# Autodesk Inventor assembly: Drive Roller Assembly 3 (Lexan)
(part 2 of 2)
- Mate:1213: Vex Pro 1x1 rectangular tubing 21.375 in length:1 ↔ Roller Crossbar Gusset (Custom):6
- Mate:1214: Vex Pro 1x1 rectangular tubing 14 in length (roller):1 ↔ Roller Crossbar Gusset (Custom):7
- Mate:1215: Vex Pro 1x1 rectangular tubing 14 in length (roller):1 ↔ Roller Crossbar Gusset (Custom):7
- Mate:1216: Vex Pro 1x1 rectangular tubing 14 in length (roller):1 ↔ Roller Crossbar Gusset (Custom):7
- Mate:1218: Vex Pro 1x1 rectangular tubing 14 in length:5 ↔ Bearing Mount Spacer 1-8 in:1
- Mate:1219: Vex Pro 1x1 rectangular tubing 14 in length:5 ↔ Bearing Mount Spacer 1-8 in:1
- Mate:1220: Vex Pro 1x1 rectangular tubing 14 in length:5 ↔ Bearing Mount Spacer 1-8 in:1
- Mate:1221: Vex Pro End Bearing Mount (Bolt):1 ↔ Bearing Mount Spacer 1-8 in:1
- Mate:1222: Vex Pro End Bearing Mount (Bolt):1 ↔ Bearing Mount Spacer 1-8 in:1
- Mate:1223: Vex Pro End Bearing Mount (Bolt):1 ↔ Bearing Mount Spacer 1-8 in:1
- Mate:1224: Vex Pro 1x1 rectangular tubing 14 in length:5 ↔ Bearing Mount Spacer 1-8 in:2
- Mate:1225: Vex Pro 1x1 rectangular tubing 14 in length:5 ↔ Bearing Mount Spacer 1-8 in:2
- Mate:1226: Vex Pro 1x1 rectangular tubing 14 in length:5 ↔ Bearing Mount Spacer 1-8 in:2
- Mate:1227: Vex Pro End Bearing Mount (Bolt):2 ↔ Bearing Mount Spacer 1-8 in:2
- Mate:1228: Vex Pro End Bearing Mount (Bolt):2 ↔ Bearing Mount Spacer 1-8 in:2
- Mate:1229: Vex Pro End Bearing Mount (Bolt):2 ↔ Bearing Mount Spacer 1-8 in:2
- Mate:1230: Vex Pro 1x1 rectangular tubing 14 in length:6 ↔ Bearing Mount Spacer 1-8 in:3
- Mate:1231: Vex Pro 1x1 rectangular tubing 14 in length:6 ↔ Bearing Mount Spacer 1-8 in:3
- Mate:1232: Vex Pro 1x1 rectangular tubing 14 in length:6 ↔ Bearing Mount Spacer 1-8 in:3
- Mate:1233: Vex Pro End Bearing Mount (Bolt):3 ↔ Bearing Mount Spacer 1-8 in:3
- Mate:1234: Vex Pro End Bearing Mount (Bolt):3 ↔ Bearing Mount Spacer 1-8 in:3
- Mate:1235: Vex Pro End Bearing Mount (Bolt):3 ↔ Bearing Mount Spacer 1-8 in:3
- Mate:1236: Vex Pro 1x1 rectangular tubing 14 in length:6 ↔ Bearing Mount Spacer 1-8 in:5
- Mate:1237: Vex Pro 1x1 rectangular tubing 14 in length:6 ↔ Bearing Mount Spacer 1-8 in:5
- Mate:1238: Vex Pro 1x1 rectangular tubing 14 in length:6 ↔ Bearing Mount Spacer 1-8 in:5
- Mate:1239: Vex Pro End Bearing Mount (Bolt):4 ↔ Bearing Mount Spacer 1-8 in:5
- Mate:1240: Vex Pro End Bearing Mount (Bolt):4 ↔ Bearing Mount Spacer 1-8 in:5
- Mate:1241: Vex Pro End Bearing Mount (Bolt):4 ↔ Bearing Mount Spacer 1-8 in:5
- Mate:1242: Hex Shaft Collar 3-8 in (7552K300):1 ↔ Hex Shaft 3-8 in (am-0855):3
- Mate:1243: Hex Shaft Collar 3-8 in (7552K300):1 ↔ Hex Shaft 3-8 in (am-0855):3
- Flush:41: Hex Shaft Collar 3-8 in (7552K300):1 ↔ Hex Shaft 3-8 in (am-0855):3
- Mate:1244: Hex Shaft Collar 3-8 in (7552K300):3 ↔ Hex Shaft 3-8 in (am-0855):4
- Mate:1245: Hex Shaft Collar 3-8 in (7552K300):3 ↔ Hex Shaft 3-8 in (am-0855):4
- Flush:42: Hex Shaft Collar 3-8 in (7552K300):3 ↔ Hex Shaft 3-8 in (am-0855):4
- Mate:1246: Vex Pro 1x1 rectangular tubing 14 in length:5 ↔ Vex Pro T gusset - OUT OF STOCK 1192014:3
- Mate:1247: Vex Pro 1x1 rectangular tubing 14 in length:5 ↔ Vex Pro T gusset - OUT OF STOCK 1192014:3
- Mate:1248: Vex Pro 1x1 rectangular tubing 14 in length:5 ↔ Vex Pro T gusset - OUT OF STOCK 1192014:3
- Mate:1249: Vex Pro 1x1 rectangular tubing 4 in length:1 ↔ Vex Pro T gusset - OUT OF STOCK 1192014:3
- Mate:1250: Vex Pro 1x1 rectangular tubing 14 in length:5 ↔ Vex Pro T gusset - OUT OF STOCK 1192014:4
- Mate:1251: Vex Pro 1x1 rectangular tubing 14 in length:5 ↔ Vex Pro T gusset - OUT OF STOCK 1192014:4
- Mate:1252: Vex Pro 1x1 rectangular tubing 14 in length:5 ↔ Vex Pro T gusset - OUT OF STOCK 1192014:4
- Mate:1253: Vex Pro 1x1 rectangular tubing 4 in length:1 ↔ Vex Pro T gusset - OUT OF STOCK 1192014:4
- Mate:1254: Vex Pro 1x1 rectangular tubing 14 in length:6 ↔ Vex Pro T gusset - OUT OF STOCK 1192014:5
- Mate:1255: Vex Pro 1x1 rectangular tubing 14 in length:6 ↔ Vex Pro T gusset - OUT OF STOCK 1192014:5
- Mate:1256: Vex Pro 1x1 rectangular tubing 14 in length:6 ↔ Vex Pro T gusset - OUT OF STOCK 1192014:5
- Mate:1257: Vex Pro 1x1 rectangular tubing 4 in length:2 ↔ Vex Pro T gusset - OUT OF STOCK 1192014:5
- Mate:1258: Vex Pro 1x1 rectangular tubing 4 in length:1 ↔ Vex Pro T gusset - OUT OF STOCK 1192014:3
- Mate:1259: Vex Pro 1x1 rectangular tubing 4 in length:2 ↔ Vex Pro T gusset - OUT OF STOCK 1192014:5
- Mate:1260: Vex Pro 1x1 rectangular tubing 14 in length:6 ↔ Vex Pro T gusset - OUT OF STOCK 1192014:6
- Mate:1261: Vex Pro 1x1 rectangular tubing 14 in length:6 ↔ Vex Pro T gusset - OUT OF STOCK 1192014:6
- Mate:1262: Vex Pro 1x1 rectangular tubing 14 in length:6 ↔ Vex Pro T gusset - OUT OF STOCK 1192014:6
- Mate:1263: Vex Pro 1x1 rectangular tubing 4 in length:2 ↔ Vex Pro T gusset - OUT OF STOCK 1192014:6
- Mate:1264: Vex Pro 1x1 rectangular tubing 4 in length:2 ↔ Vex Pro T gusset - OUT OF STOCK 1192014:6
- Mate:1265: Vex Pro 1x1 rectangular tubing 4 in length:1 ↔ Vex Pro T gusset - OUT OF STOCK 1192014:3
- Mate:1266: Hex Spacer:3 ↔ Clamp with Piston Assembly (new):1
- Mate:1267: Vex Pro 1x1 rectangular tubing 21.375 in length:1 ↔ Roller Crossbar Gusset (Custom):5
- Mate:1268: Vex Pro 1x1 rectangular tubing 21.375 in length:1 ↔ Roller Crossbar Gusset (Custom):5
- Mate:1269: Vex Pro 1x1 rectangular tubing 21.375 in length:1 ↔ Roller Crossbar Gusset (Custom):5
- Mate:1270: Pneumatic Piston Front Flange (Rt Custom):2 ↔ Clamp Piston ( 1 in stroke twice, 9-16 bore):1
- Mate:1271: Pneumatic Piston Front Flange (Lt Custom):1 ↔ Clamp Piston ( 1 in stroke twice, 9-16 bore):2
- Mate:1272: Vex Pro 1x1 rectangular tubing 14 in length:5 ↔ Roller Piston 4 Mount:1
- Mate:1273: Vex Pro 1x1 rectangular tubing 14 in length:5 ↔ Roller Piston 4 Mount:1
- Mate:1274: Vex Pro 1x1 rectangular tubing 14 in length:5 ↔ Roller Piston 4 Mount:1
- Mate:1275: Vex Pro 1x1 rectangular tubing 14 in length:6 ↔ Roller Piston 4 Mount:2
- Mate:1276: Vex Pro 1x1 rectangular tubing 14 in length:6 ↔ Roller Piston 4 Mount:2
- Mate:1277: Vex Pro 1x1 rectangular tubing 14 in length:6 ↔ Roller Piston 4 Mount:2
- Mate:1278: Roller Piston 4 Mount:2 ↔ Roller Piston 4 (.5 and 1 in Stroke, 9-16 in Bore):1
- Mate:1279: Roller Piston 4 Mount:2 ↔ Roller Piston 4 (.5 and 1 in Stroke, 9-16 in Bore):1
- Mate:1280: Roller Piston 4 Mount:1 ↔ Roller Piston 4 (.5 and 1 in Stroke, 9-16 in Bore):2
- Mate:1281: Roller Piston 4 Mount:1 ↔ Roller Piston 4 (.5 and 1 in Stroke, 9-16 in Bore):2
- Mate:1282: Bracket:3 ↔ Roller Piston 4 (.5 and 1 in Stroke, 9-16 in Bore):2
- Mate:1283: Shaft Collar 3-16 in ID (6435K510):2 ↔ Roller Piston 4 (.5 and 1 in Stroke, 9-16 in Bore):2
- Mate:1284: Shaft Collar 3-16 in ID (6435K510):1 ↔ Roller Piston 4 (.5 and 1 in Stroke, 9-16 in Bore):2
- Mate:1285: Bracket:4 ↔ Roller Piston 4 (.5 and 1 in Stroke, 9-16 in Bore):1
- Mate:1286: Shaft Collar 3-16 in ID (6435K510):4 ↔ Roller Piston 4 (.5 and 1 in Stroke, 9-16 in Bore):1
- Mate:1287: Shaft Collar 3-16 in ID (6435K510):3 ↔ Roller Piston 4 (.5 and 1 in Stroke, 9-16 in Bore):1
- Mate:1288: Vex Pro 1x1 rectangular tubing 4 in length:3 ↔ Vex Pro T gusset - OUT OF STOCK 1192014:1
- Mate:1289: Vex Pro 1x1 rectangular tubing 14 in length:6 ↔ Vex Pro T gusset - OUT OF STOCK 1192014:7
- Mate:1290: Vex Pro 1x1 rectangular tubing 14 in length:6 ↔ Vex Pro T gusset - OUT OF STOCK 1192014:7
- Mate:1291: Vex Pro 1x1 rectangular tubing 14 in length:6 ↔ Vex Pro T gusset - OUT OF STOCK 1192014:7
- Mate:1292: Vex Pro 1x1 rectangular tubing 14 in length:6 ↔ Vex Pro T gusset - OUT OF STOCK 1192014:8
- Mate:1293: Vex Pro 1x1 rectangular tubing 14 in length:6 ↔ Vex Pro T gusset - OUT OF STOCK 1192014:8
- Mate:1294: Vex Pro 1x1 rectangular tubing 14 in length:6 ↔ Vex Pro T gusset - OUT OF STOCK 1192014:8
- Mate:1295: Vex Pro T gusset - OUT OF STOCK 1192014:8 ↔ Vex Pro 1x1 rectangular tubing 4 in length:4
- Mate:1296: Vex Pro T gusset - OUT OF STOCK 1192014:7 ↔ Vex Pro 1x1 rectangular tubing 4 in length:4
- Mate:1297: Vex Pro T gusset - OUT OF STOCK 1192014:7 ↔ Vex Pro 1x1 rectangular tubing 4 in length:4
- Mate:1298: Vex Pro T gusset - OUT OF STOCK 1192014:8 ↔ Vex Pro 1x1 rectangular tubing 2 in length (no hex):2
- Mate:1299: Vex Pro T gusset - OUT OF STOCK 1192014:7 ↔ Vex Pro 1x1 rectangular tubing 2 in length (no hex):2
- Flush:43: Vex Pro T gusset - OUT OF STOCK 1192014:7 ↔ Vex Pro 1x1 rectangular tubing 2 in length (no hex):2
## Named parameters: d240_d195 = 0 mm, d241_d196 = 0 mm, d242_d197 = 0 mm, d243_d198 = 0 mm, d305_d302 = 0 mm, d306_d303 = 0 mm, d307_d304 = 0 mm, d334_d317 = 0 mm, d339_d304 = 0 mm, d343_d308 = 0 mm, d344_d309 = 0 mm, d345_d310 = 0 mm, d346_d316 = 0 mm, d349_d328 = 0 mm, d350_d329 = 0 mm, d352_d331 = 0 mm, d353_d332 = 0 mm, d770_d743 = 0 mm, d771_d744 = 0 mm, d772_d745 = 0 mm, d773_d746 = 0 mm, d791_d742 = 0 mm, d1331_d1327 = 0 mm, d1332_d1328 = 0 mm, d1398_d1387 = 0 mm, d1399_d1388 = 0 mm, d1400_d1389 = 0 mm, d1404_d1384 = 0 mm, d1405_d1385 = 0 mm, d1406_d1386 = 0 mm
